# Autodesk Inventor assembly: Assembly1
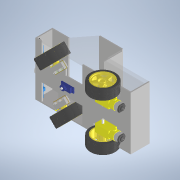
[picture p0: Inventor's stored thumbnail of the model, 180x180]
Saved by Autodesk Inventor 2022 (Build 260153000, 153)
## iProperties
Created: 2021-12-16
Part Number: Assembly1
Document SubType Name: Assembly
Designer: keemi
Author: keemi
## Documents named in this file (9)
- C:\Users\keemi\OneDrive\Bureaublad\repo's\projecten\Auto\modellen\inventor\auto moddel\Assembly1.iam
- C:\Users\keemi\OneDrive\Bureaublad\repo's\projecten\Auto\modellen\inventor\auto moddel\zijkant.ipt
- C:\Users\keemi\OneDrive\Bureaublad\repo's\projecten\Auto\modellen\inventor\auto moddel\voorkant.ipt
- C:\Users\keemi\OneDrive\Bureaublad\repo's\projecten\Auto\modellen\inventor\auto moddel\achterkant.ipt
- C:\Users\keemi\OneDrive\Bureaublad\repo's\projecten\Auto\modellen\inventor\auto moddel\motorkap.ipt
- C:\Users\keemi\OneDrive\Bureaublad\repo's\projecten\Auto\modellen\inventor\auto moddel\achterruit.ipt
- C:\Users\keemi\OneDrive\Bureaublad\repo's\projecten\Auto\modellen\inventor\auto moddel\bak.ipt
- C:\Users\keemi\OneDrive\Bureaublad\repo's\projecten\Auto\modellen\inventor\auto moddel\DAK.ipt
- C:\Users\keemi\OneDrive\Bureaublad\repo's\projecten\Auto\modellen\inventor\auto moddel\ONDERPLAAT.iam
## Components (9 placed, 8 different names)
1. zijkant:1 — Flush:13, Flush:14, Flush:15, Flush:16, Flush:18, Flush:20, Flush:24, Flush:27, Flush:28, Flush:29
2. zijkant:2 — Flush:9, Flush:10, Mate:1, Flush:23, Flush:25, Flush:30, Flush:32
3. voorkant:1 — Flush:9, Flush:10, Flush:13, Flush:17, Flush:19, Flush:31
4. achterkant:1 — Flush:14, Flush:15, Flush:16
5. motorkap:1 — Flush:17, Flush:18, Flush:19
6. achterruit:1 — Flush:20, Flush:21, Flush:22, Flush:23, Flush:26
7. bak:1 — Flush:21, Flush:22, Mate:1
8. DAK:1 — Flush:24, Flush:25, Flush:26
9. ONDERPLAAT:1 [sub-assembly] — Flush:27, Flush:28, Flush:29, Flush:30, Flush:31, Flush:32
## Relationships (23: Flush 22, Mate 1)
- Flush:9: zijkant:2 ↔ voorkant:1
- Flush:10: zijkant:2 ↔ voorkant:1
- Flush:13: zijkant:1 ↔ voorkant:1
- Flush:14: zijkant:1 ↔ achterkant:1
- Flush:15: zijkant:1 ↔ achterkant:1
- Flush:16: zijkant:1 ↔ achterkant:1
- Flush:17: voorkant:1 ↔ motorkap:1
- Flush:18: zijkant:1 ↔ motorkap:1
- Flush:19: voorkant:1 ↔ motorkap:1
- Flush:20: zijkant:1 ↔ achterruit:1
- Flush:21: achterruit:1 ↔ bak:1
- Flush:22: achterruit:1 ↔ bak:1
- Mate:1: zijkant:2 ↔ bak:1
- Flush:23: zijkant:2 ↔ achterruit:1
- Flush:24: zijkant:1 ↔ DAK:1
- Flush:25: zijkant:2 ↔ DAK:1
- Flush:26: achterruit:1 ↔ DAK:1
- Flush:27: zijkant:1 ↔ ONDERPLAAT:1
- Flush:28: zijkant:1 ↔ ONDERPLAAT:1
- Flush:29: zijkant:1 ↔ ONDERPLAAT:1
- Flush:30: zijkant:2 ↔ ONDERPLAAT:1
- Flush:31: voorkant:1 ↔ ONDERPLAAT:1
- Flush:32: zijkant:2 ↔ ONDERPLAAT:1
